# Autodesk Inventor assembly: drive encoder assembly
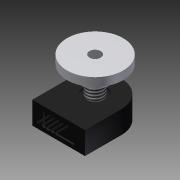
[picture p0: Inventor's stored thumbnail of the model, 180x180]
Saved by Autodesk Inventor 2012 (Build 160160000, 160)
## iProperties
Created: 2012-07-13
Part Number: drive encoder assembly
Document SubType Name: Assembly
Designer: Bryce
Author: Bryce
## Documents named in this file (3)
- C:\Users\Bryce\Dropbox\Inventor Design Project Files\Independent Swerves\Inventor 2012\drive encoder assembly.iam
- C:\Users\Bryce\Dropbox\Inventor Design Project Files\Independent Swerves\Imported Components\Encoder USD S1-100-B Assy.iam
- C:\Users\Bryce\Dropbox\Inventor Design Project Files\Independent Swerves\Imported Components\a_1m_2-y24054\a_1m_2-y24054 3.ipt
## Components (2 placed, 2 different names)
1. Encoder USD S1-100-B Assy:1 [sub-assembly] — Mate:5, Mate:6
2. a_1m_2-y24054 3:1 — Mate:5, Mate:6
## Relationships (2: Mate 2)
- Mate:5 (1.5875 mm): Encoder USD S1-100-B Assy:1 ↔ a_1m_2-y24054 3:1
- Mate:6: Encoder USD S1-100-B Assy:1 ↔ a_1m_2-y24054 3:1
